# Autodesk Inventor assembly: FollowAlongAssembly
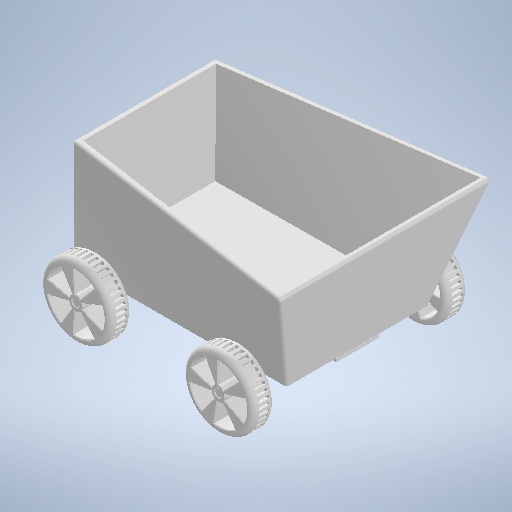
[picture p0: Inventor's stored thumbnail of the model, 512x512]
Saved by Autodesk Inventor 2025.1 (Build 291241020, 241B)
## iProperties
Created: 2024-12-27
Part Number: FollowAlongAssembly
Document SubType Name: Assembly
Designer: herme
Author: herme
## Documents named in this file (4)
- C:\Users\herme\Documents\Sumobot\CAD\FollowAlongAssembly.iam
- C:\Users\herme\Documents\Sumobot\CAD\AssemblyFiles\base_and_axels.ipt
- C:\Users\herme\Documents\Sumobot\CAD\AssemblyFiles\trolley_body.ipt
- C:\Users\herme\Documents\Sumobot\CAD\AssemblyFiles\wheel.ipt
## Components (6 placed, 3 different names)
1. base_and_axels:1 — Insert:1, Insert:2, Insert:3, Insert:4, Mate:1, Mate:2, Mate:3
2. trolley_body:1 — Mate:1, Mate:2, Mate:3
3. wheel:1 — Insert:1
4. wheel:2 — Insert:3
5. wheel:3 — Insert:4
6. wheel:4 — Insert:2
## Relationships (7: Insert 4, Mate 3)
- Insert:1: base_and_axels:1 ↔ wheel:1
- Insert:2: base_and_axels:1 ↔ wheel:4
- Insert:3: base_and_axels:1 ↔ wheel:2
- Insert:4: base_and_axels:1 ↔ wheel:3
- Mate:1: base_and_axels:1 ↔ trolley_body:1
- Mate:2: base_and_axels:1 ↔ trolley_body:1
- Mate:3: base_and_axels:1 ↔ trolley_body:1
